# Autodesk Inventor assembly: Cooling Camber 2 inventor
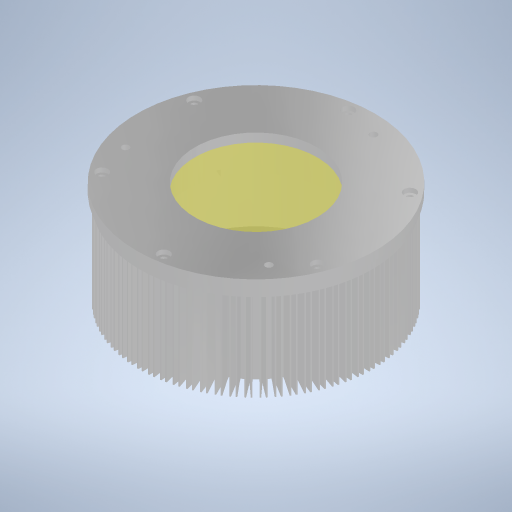
[picture p0: Inventor's stored thumbnail of the model, 512x512]
Saved by Autodesk Inventor 2023 (Build 270158000, 158)
## iProperties
Created: 2024-03-16
Part Number: Cooling Camber 2 inventor
Document SubType Name: Assembly
Designer: test
Author: test
## Documents named in this file (4)
- D:\Mount Project\Cooler DSLR\CNC Fixed\Cooling Camber 2 inventor.iam
- D:\Mount Project\Cooler DSLR\CNC Fixed\Filter Kaca.ipt
- D:\Mount Project\Cooler DSLR\CNC Fixed\Peltier.ipt
- D:\Mount Project\Cooler DSLR\CNC Fixed\Cooling Camber tanpa kacaa.ipt
## Components (3 placed, 3 different names)
1. Filter Kaca:1 — Rotational:1
2. Peltier:1 — Rigid:1
3. Cooling Camber tanpa kacaa:1 — Rotational:1, Rigid:1
## Relationships (2: RevoluteJoint 1, WeldJoint 1)
- Rotational:1 [RevoluteJoint]: Filter Kaca:1 ↔ Cooling Camber tanpa kacaa:1
- Rigid:1 [WeldJoint]: Peltier:1 ↔ Cooling Camber tanpa kacaa:1
